# Autodesk Inventor assembly: Gripper General
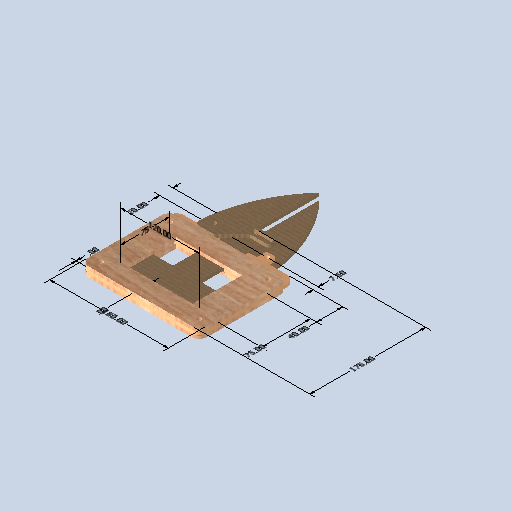
[picture p0: Inventor's stored thumbnail of the model, 512x512]
Saved by Autodesk Inventor 2023.1 (Build 271208000, 208)
## iProperties
Created: 2022-11-11
Part Number: Gripper General
Document SubType Name: Assembly
Designer: Daniel Peña
Author: Daniel Peña
## Documents named in this file (6)
- C:\Users\danie\Documents\UN\ProyectoRobotica\CAD\V3 - BigChungus\Gripper General.iam
- C:\Users\danie\Documents\UN\ProyectoRobotica\CAD\V3 - BigChungus\MarcoBC.ipt
- C:\Users\danie\Documents\UN\ProyectoRobotica\CAD\V3 - BigChungus\PistonBC.ipt
- C:\Users\danie\Documents\UN\ProyectoRobotica\CAD\V3 - BigChungus\Dedo-BC.ipt
- C:\Users\danie\Documents\UN\ProyectoRobotica\CAD\V3 - BigChungus\TapaBC.ipt
- C:\Users\danie\Documents\UN\ProyectoRobotica\CAD\PortaHerramienta\Ventosa.ipt
## Components (7 placed, 5 different names)
1. MarcoBC:1 — Slider:1, Rotational:1, Rotational:2, Insert:1, Insert:2, Insert:3, Insert:4, Insert:5, Insert:6, Insert:7, Insert:8
2. PistonBC:1 — Slider:1, Tangent:1, Tangent:2
3. Dedo-BC:1 — Rotational:2, Tangent:1
4. Dedo-BC:2 — Rotational:1, Tangent:2
5. TapaBC:1 — Insert:5, Insert:6, Insert:7, Insert:8
6. Ventosa:1
7. TapaBC:2 — Insert:1, Insert:2, Insert:3, Insert:4
## Relationships (13: Insert 8, RevoluteJoint 2, Tangent 2, TranslationJoint 1)
- Slider:1 [TranslationJoint]: MarcoBC:1 ↔ PistonBC:1
- Rotational:1 [RevoluteJoint]: MarcoBC:1 ↔ Dedo-BC:2
- Rotational:2 [RevoluteJoint]: MarcoBC:1 ↔ Dedo-BC:1
- Tangent:1: PistonBC:1 ↔ Dedo-BC:1
- Tangent:2: PistonBC:1 ↔ Dedo-BC:2
- Insert:1: MarcoBC:1 ↔ TapaBC:2
- Insert:2: MarcoBC:1 ↔ TapaBC:2
- Insert:3: MarcoBC:1 ↔ TapaBC:2
- Insert:4: MarcoBC:1 ↔ TapaBC:2
- Insert:5: MarcoBC:1 ↔ TapaBC:1
- Insert:6: MarcoBC:1 ↔ TapaBC:1
- Insert:7: MarcoBC:1 ↔ TapaBC:1
- Insert:8: MarcoBC:1 ↔ TapaBC:1
